# Autodesk Inventor assembly: Dehoanthanh
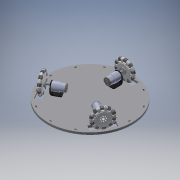
[picture p0: Inventor's stored thumbnail of the model, 180x180]
Saved by Autodesk Inventor 2019 (Build 230136000, 136)
## iProperties
Created: 2021-01-20
Part Number: Dehoanthanh
Document SubType Name: Assembly
Designer: Admin
Author: Admin
## Documents named in this file (3)
- C:\Users\Admin\Documents\Inventor\Doan\Dehoanthanh.iam
- C:\Users\Admin\Documents\Inventor\Doan\Banhxenew.iam
- C:\Users\Admin\Documents\Inventor\Doan\denew.ipt
## Components (4 placed, 2 different names)
1. denew:1 — Mate:1, Mate:2, Mate:3
2. Banhxenew:1 [sub-assembly] — Mate:1, Mate:2, Mate:3
3. Banhxenew:2 [sub-assembly]
4. Banhxenew:3 [sub-assembly]
## Component patterns: (3 elements, first: Banhxenew:1)
## Relationships (3: Mate 3)
- Mate:1: denew:1 ↔ Banhxenew:1
- Mate:2: denew:1 ↔ Banhxenew:1
- Mate:3: denew:1 ↔ Banhxenew:1
